# Autodesk Inventor assembly: Alex_holder
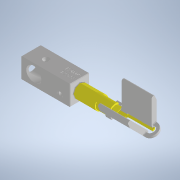
[picture p0: Inventor's stored thumbnail of the model, 180x180]
Saved by Autodesk Inventor 2022 (Build 260153000, 153)
## iProperties
Created: 2022-08-26
Part Number: Alex_holder
Document SubType Name: Assembly
Designer: Daniel
Author: Daniel
## Documents named in this file (4)
- E:\OneDrive - Imperial College London\DragonVision_DanielKo\Instrumentation\Ephys_rig_2021\Holder\Alex_holder.iam
- E:\OneDrive - Imperial College London\DragonVision_DanielKo\Instrumentation\Ephys_rig_2021\Holder\holderHolder.ipt
- E:\OneDrive - Imperial College London\DragonVision_DanielKo\Instrumentation\Ephys_rig_2021\Holder\body_adjustable_parametric_v3.ipt
- E:\OneDrive - Imperial College London\DragonVision_DanielKo\Instrumentation\Ephys_rig_2021\Holder\alex_dorsal_v4.ipt
## Components (3 placed, 3 different names)
1. holderHolder:1 — Mate:1, asdqwd
2. body_adjustable_parametric_v3:1 — Mate:1, asdqwd, Mate:2, Mate:3, Mate:4
3. alex_dorsal_v4:1 — Mate:2, Mate:3, Mate:4
## Relationships (5: Mate 4, Angle 1)
- Mate:1: holderHolder:1 ↔ body_adjustable_parametric_v3:1
- asdqwd [Angle] (270 deg): holderHolder:1 ↔ body_adjustable_parametric_v3:1
- Mate:2: body_adjustable_parametric_v3:1 ↔ alex_dorsal_v4:1
- Mate:3: body_adjustable_parametric_v3:1 ↔ alex_dorsal_v4:1
- Mate:4: body_adjustable_parametric_v3:1 ↔ alex_dorsal_v4:1
